# Autodesk Inventor assembly: Track Frame Assembly
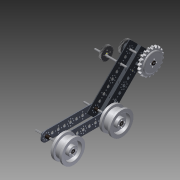
[picture p0: Inventor's stored thumbnail of the model, 180x180]
Saved by Autodesk Inventor 2015 (Build 190159000, 159)
## iProperties
Created: 2015-09-27
Part Number: Track Frame Assembly
Document SubType Name: Assembly
Designer: Jing-Chen
Author: Jing-Chen
## Documents named in this file (11)
- C:\Users\Jing-Chen\Desktop\Bionic Hybrids 2016\Bionic-Hybrids\CAD\Drivetrain\Sub-Assemblies\Track Frame Assembly.iam
- C:\Users\Jing-Chen\Desktop\Bionic Hybrids 2016\Bionic-Hybrids\Stock\Bracket-U9 - 739067.ipt
- C:\Users\Jing-Chen\Desktop\Bionic Hybrids 2016\Bionic-Hybrids\CAD\Drivetrain\Sub-Assemblies\Track Idler Assembly.iam
- C:\Users\Jing-Chen\Desktop\Bionic Hybrids 2016\Bionic-Hybrids\Stock\Axle-100mm - 739088.ipt
- C:\Users\Jing-Chen\Desktop\Bionic Hybrids 2016\Bionic-Hybrids\Stock\Bearing-Thrust - 739091.ipt
- C:\Users\Jing-Chen\Desktop\Bionic Hybrids 2016\Bionic-Hybrids\Stock\Shaft Collar-Setscrew, Axle - 739092.iam
- C:\Users\Jing-Chen\Desktop\Bionic Hybrids 2016\Bionic-Hybrids\Stock\Track Sprocket - 736468.ipt
- C:\Users\Jing-Chen\Desktop\Bionic Hybrids 2016\Bionic-Hybrids\Stock\Shaft Collar-Setscrew, Axle, Mountable - 739172.iam
- C:\Users\Jing-Chen\Desktop\Bionic Hybrids 2016\Bionic-Hybrids\Stock\Plate-9x1 - 739272.ipt
- C:\Users\Jing-Chen\Desktop\Bionic Hybrids 2016\Bionic-Hybrids\Stock\Spacer 3.125mm- 739100.ipt
- C:\Users\Jing-Chen\Desktop\Bionic Hybrids 2016\Bionic-Hybrids\Stock\Gear-40 tooth - 731901.ipt
## Components (25 placed, 10 different names)
1. Bracket-U9 - 739067:1 — Mate:5, Mate:16, Mate:17, Mate:18, Mate:19, Mate:20, Mate:21, Mate:34, Mate:44, Mate:46, Mate:60, Mate:61, Mate:63, Flush:6, Mate:66
2. Track Idler Assembly:1 [sub-assembly] — Mate:2, Flush:1, Mate:43
3. Axle-100mm - 739088:1 — Mate:2, Flush:1, Mate:11, Mate:41
4. Bearing-Thrust - 739091:2 — Mate:5, Mate:31, Mate:36, Mate:62
5. Shaft Collar-Setscrew, Axle - 739092:1 [sub-assembly] — Mate:11, Mate:42
6. Track Sprocket - 736468:1 — Mate:13, Mate:14, Mate:15, Mate:23, Mate:24
7. Shaft Collar-Setscrew, Axle, Mountable - 739172:1 [sub-assembly] — Mate:13, Mate:14, Mate:15, Mate:22, Mate:31
8. Plate-9x1 - 739272:1 — Mate:16, Mate:19, Mate:21, Mate:37, Mate:38, Mate:45, Flush:4, Flush:5, Mate:53
9. Plate-9x1 - 739272:2 — Mate:17, Mate:18, Mate:20, Mate:39, Mate:40, Mate:47
10. Axle-100mm - 739088:2 — Mate:22, Flush:2, Mate:33, Mate:35, Mate:58, Mate:62
11. Bearing-Thrust - 739091:4 — Mate:23, Mate:24, Flush:2
12. Spacer 3.125mm- 739100:1 — Mate:32, Mate:33, Mate:34
13. Spacer 3.125mm- 739100:2 — Mate:32, Mate:35, Mate:36
14. Bearing-Thrust - 739091:5 — Mate:44, Mate:45, Mate:48, Mate:50
15. Bearing-Thrust - 739091:6 — Mate:39, Mate:40, Mate:41, Mate:42
16. Bearing-Thrust - 739091:10 — Mate:46, Mate:47, Mate:52
17. Bearing-Thrust - 739091:11 — Mate:37, Mate:38, Mate:43
18. Axle-100mm - 739088:3 — Mate:48, Mate:49, Flush:3, Mate:51
19. Track Idler Assembly:2 [sub-assembly] — Mate:49, Mate:50, Flush:3
20. Shaft Collar-Setscrew, Axle - 739092:2 [sub-assembly] — Mate:51, Mate:52
21. Gear-40 tooth - 731901:1 — Mate:55, Mate:57, Mate:64
22. Gear-40 tooth - 731901:2
23. Shaft Collar-Setscrew, Axle, Mountable - 739172:2 [sub-assembly] — Mate:55, Mate:57, Mate:58, Mate:63, Mate:64
24. Shaft Collar-Setscrew, Axle, Mountable - 739172:4 [sub-assembly] — Mate:60, Mate:61, Mate:65, Mate:66
25. Axle-100mm - 739088:4 — Mate:65, Flush:6
## Relationships (54: Mate 48, Flush 6)
- Mate:2: Track Idler Assembly:1 ↔ Axle-100mm - 739088:1
- Mate:5: Bracket-U9 - 739067:1 ↔ Bearing-Thrust - 739091:2
- Flush:1: Track Idler Assembly:1 ↔ Axle-100mm - 739088:1
- Mate:11: Axle-100mm - 739088:1 ↔ Shaft Collar-Setscrew, Axle - 739092:1
- Mate:13: Track Sprocket - 736468:1 ↔ Shaft Collar-Setscrew, Axle, Mountable - 739172:1
- Mate:14: Track Sprocket - 736468:1 ↔ Shaft Collar-Setscrew, Axle, Mountable - 739172:1
- Mate:15: Track Sprocket - 736468:1 ↔ Shaft Collar-Setscrew, Axle, Mountable - 739172:1
- Mate:16: Bracket-U9 - 739067:1 ↔ Plate-9x1 - 739272:1
- Mate:17: Bracket-U9 - 739067:1 ↔ Plate-9x1 - 739272:2
- Mate:18: Bracket-U9 - 739067:1 ↔ Plate-9x1 - 739272:2
- Mate:19: Bracket-U9 - 739067:1 ↔ Plate-9x1 - 739272:1
- Mate:20: Bracket-U9 - 739067:1 ↔ Plate-9x1 - 739272:2
- Mate:21: Bracket-U9 - 739067:1 ↔ Plate-9x1 - 739272:1
- Mate:22: Shaft Collar-Setscrew, Axle, Mountable - 739172:1 ↔ Axle-100mm - 739088:2
- Mate:23: Track Sprocket - 736468:1 ↔ Bearing-Thrust - 739091:4
- Mate:24: Track Sprocket - 736468:1 ↔ Bearing-Thrust - 739091:4
- Flush:2: Axle-100mm - 739088:2 ↔ Bearing-Thrust - 739091:4
- Mate:31: Bearing-Thrust - 739091:2 ↔ Shaft Collar-Setscrew, Axle, Mountable - 739172:1
- Mate:32: Spacer 3.125mm- 739100:1 ↔ Spacer 3.125mm- 739100:2
- Mate:33: Axle-100mm - 739088:2 ↔ Spacer 3.125mm- 739100:1
- Mate:34: Bracket-U9 - 739067:1 ↔ Spacer 3.125mm- 739100:1
- Mate:35: Axle-100mm - 739088:2 ↔ Spacer 3.125mm- 739100:2
- Mate:36: Bearing-Thrust - 739091:2 ↔ Spacer 3.125mm- 739100:2
- Mate:37: Plate-9x1 - 739272:1 ↔ Bearing-Thrust - 739091:11
- Mate:38: Plate-9x1 - 739272:1 ↔ Bearing-Thrust - 739091:11
- Mate:39: Plate-9x1 - 739272:2 ↔ Bearing-Thrust - 739091:6
- Mate:40: Plate-9x1 - 739272:2 ↔ Bearing-Thrust - 739091:6
- Mate:41: Axle-100mm - 739088:1 ↔ Bearing-Thrust - 739091:6
- Mate:42: Shaft Collar-Setscrew, Axle - 739092:1 ↔ Bearing-Thrust - 739091:6
- Mate:43: Track Idler Assembly:1 ↔ Bearing-Thrust - 739091:11
- Mate:44: Bracket-U9 - 739067:1 ↔ Bearing-Thrust - 739091:5
- Mate:45: Plate-9x1 - 739272:1 ↔ Bearing-Thrust - 739091:5
- Mate:46: Bracket-U9 - 739067:1 ↔ Bearing-Thrust - 739091:10
- Mate:47: Plate-9x1 - 739272:2 ↔ Bearing-Thrust - 739091:10
- Mate:48: Bearing-Thrust - 739091:5 ↔ Axle-100mm - 739088:3
- Mate:49: Axle-100mm - 739088:3 ↔ Track Idler Assembly:2
- Mate:50: Bearing-Thrust - 739091:5 ↔ Track Idler Assembly:2
- Flush:3: Axle-100mm - 739088:3 ↔ Track Idler Assembly:2
- Mate:51: Axle-100mm - 739088:3 ↔ Shaft Collar-Setscrew, Axle - 739092:2
- Mate:52: Bearing-Thrust - 739091:10 ↔ Shaft Collar-Setscrew, Axle - 739092:2
- Flush:4: Plate-9x1 - 739272:1
- Flush:5: Plate-9x1 - 739272:1
- Mate:53: Plate-9x1 - 739272:1
- Mate:55: Gear-40 tooth - 731901:1 ↔ Shaft Collar-Setscrew, Axle, Mountable - 739172:2
- Mate:57: Gear-40 tooth - 731901:1 ↔ Shaft Collar-Setscrew, Axle, Mountable - 739172:2
- Mate:58: Axle-100mm - 739088:2 ↔ Shaft Collar-Setscrew, Axle, Mountable - 739172:2
- Mate:60: Bracket-U9 - 739067:1 ↔ Shaft Collar-Setscrew, Axle, Mountable - 739172:4
- Mate:61: Bracket-U9 - 739067:1 ↔ Shaft Collar-Setscrew, Axle, Mountable - 739172:4
- Mate:62: Bearing-Thrust - 739091:2 ↔ Axle-100mm - 739088:2
- Mate:63: Bracket-U9 - 739067:1 ↔ Shaft Collar-Setscrew, Axle, Mountable - 739172:2
- Mate:64: Gear-40 tooth - 731901:1 ↔ Shaft Collar-Setscrew, Axle, Mountable - 739172:2
- Mate:65: Shaft Collar-Setscrew, Axle, Mountable - 739172:4 ↔ Axle-100mm - 739088:4
- Flush:6: Bracket-U9 - 739067:1 ↔ Axle-100mm - 739088:4
- Mate:66: Bracket-U9 - 739067:1 ↔ Shaft Collar-Setscrew, Axle, Mountable - 739172:4
